# Autodesk Inventor assembly: assem
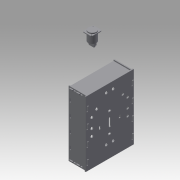
[picture p0: Inventor's stored thumbnail of the model, 180x180]
Saved by Autodesk Inventor 2019.3 (Build 233278000, 278)
## iProperties
Created: 2019-06-26
Part Number: assem
Document SubType Name: Assembly
Designer: Dave
Author: Dave
## Documents named in this file (7)
- C:\Users\Dave\Dropbox\ProjectODMeter\HousingCAD\CoilHousing\assem.iam
- C:\Users\Dave\Dropbox\ProjectODMeter\HousingCAD\CoilHousing\bottom.ipt
- C:\Users\Dave\Dropbox\ProjectODMeter\HousingCAD\CoilHousing\hdmi_recepticle_placeholder.ipt
- C:\Users\Dave\Dropbox\ProjectODMeter\HousingCAD\CoilHousing\long_side1.ipt
- C:\Users\Dave\Dropbox\ProjectODMeter\HousingCAD\CoilHousing\long_side2.ipt
- C:\Users\Dave\Dropbox\ProjectODMeter\HousingCAD\CoilHousing\shortside.ipt
- C:\Users\Dave\Dropbox\ProjectODMeter\HousingCAD\top_plate.ipt
## Components (7 placed, 6 different names)
1. bottom:1 — Mate:1, Mate:2, Mate:3, Mate:4, Mate:5, Mate:6
2. hdmi_recepticle_placeholder:1
3. long_side1:1 — Mate:1, Mate:2, Mate:3, Mate:7, Mate:8, Mate:9, Mate:10
4. long_side2:1 — Mate:4, Mate:5, Mate:6, Mate:11, Mate:12, Mate:13, Mate:14, Mate:15
5. shortside:1 — Mate:7, Mate:8, Mate:9
6. shortside:2 — Mate:10, Mate:11, Mate:12
7. top_plate:1 — Mate:13, Mate:14, Mate:15
## Relationships (15: Mate 15)
- Mate:1: bottom:1 ↔ long_side1:1
- Mate:2: bottom:1 ↔ long_side1:1
- Mate:3: bottom:1 ↔ long_side1:1
- Mate:4: bottom:1 ↔ long_side2:1
- Mate:5: bottom:1 ↔ long_side2:1
- Mate:6: bottom:1 ↔ long_side2:1
- Mate:7: long_side1:1 ↔ shortside:1
- Mate:8: long_side1:1 ↔ shortside:1
- Mate:9: long_side1:1 ↔ shortside:1
- Mate:10: long_side1:1 ↔ shortside:2
- Mate:11: long_side2:1 ↔ shortside:2
- Mate:12: long_side2:1 ↔ shortside:2
- Mate:13: long_side2:1 ↔ top_plate:1
- Mate:14: long_side2:1 ↔ top_plate:1
- Mate:15: long_side2:1 ↔ top_plate:1
